# Autodesk Inventor assembly: VP-Input-MiniCIM
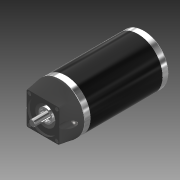
[picture p0: Inventor's stored thumbnail of the model, 180x180]
Saved by Autodesk Inventor 2022 (Build 260153000, 153)
## iProperties
Created: 2018-08-19
Part Number: VP-Input-MiniCIM
Document SubType Name: Assembly
## Documents named in this file (8)
- E:\Middleton Robotics\Collaborative Robots\Collaborative Part Library\General Gearboxes\Planetaries\Versaplanetary\V2 Stages\CIM Input Stage\VP MiniCIM Input.iam
- E:\Middleton Robotics\Collaborative Robots\Collaborative Part Library\General Gearboxes\Planetaries\Versaplanetary\Motor Mounting Plates\VP CIM Adapter.ipt
- E:\Middleton Robotics\Collaborative Robots\Collaborative Part Library\General Gearboxes\Planetaries\Versaplanetary\Input Coupler\Coupler Set Screw.ipt
- E:\Middleton Robotics\Collaborative Robots\Collaborative Part Library\General Gearboxes\Planetaries\Versaplanetary\Input Coupler\VP Input Coupler.ipt
- E:\Middleton Robotics\Collaborative Robots\Collaborative Part Library\General Gearboxes\Planetaries\Versaplanetary\Screws\10-32 x .50in Screw.ipt
- E:\Middleton Robotics\Collaborative Robots\Collaborative Part Library\Motors\FRC\Mini Cim.ipt
- E:\Middleton Robotics\Collaborative Robots\Collaborative Part Library\Motors\FRC\CIM Motor.ipt
- E:\Middleton Robotics\Collaborative Robots\Collaborative Part Library\General Gearboxes\Planetaries\Versaplanetary\V2 Stages\CIM Input Stage.iam
## Components (7 placed, 6 different names)
1. VP CIM Adapter:1 — Insert:3, Insert:4
2. CIM Motor:1
3. Coupler Set Screw:1 — Mate:3, Tangent:1
4. VP Input Coupler:1 — Mate:3, Tangent:1
5. 10-32 x .50in Screw:1 — Insert:3
6. 10-32 x .50in Screw:2 — Insert:4
7. Mini Cim:1
## Relationships (12: Insert 6, Mate 5, Tangent 1)
- [Insert]: VP CIM Adapter:1 ↔ CIM Motor:1
- [Insert]: VP CIM Adapter:1 ↔ CIM Motor:1
- [Mate]: CIM Motor:1 ↔ VP Input Coupler:1
- [Mate] (1.1 mm): CIM Motor:1 ↔ VP Input Coupler:1
- Mate:3: Coupler Set Screw:1 ↔ VP Input Coupler:1
- Tangent:1: Coupler Set Screw:1 ↔ VP Input Coupler:1
- Insert:3: VP CIM Adapter:1 ↔ 10-32 x .50in Screw:1
- Insert:4: VP CIM Adapter:1 ↔ 10-32 x .50in Screw:2
- [Insert]: VP CIM Adapter:1 ↔ Mini Cim:1
- [Insert]: VP CIM Adapter:1 ↔ Mini Cim:1
- [Mate]: VP Input Coupler:1 ↔ Mini Cim:1
- [Mate] (1.1 mm): VP Input Coupler:1 ↔ Mini Cim:1
